# Autodesk Inventor assembly: Gas
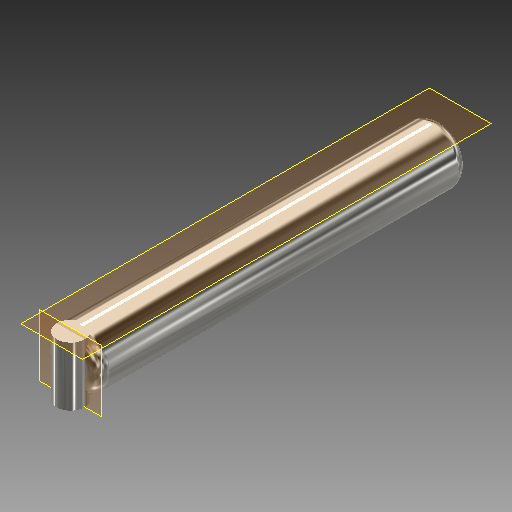
[picture p0: Inventor's stored thumbnail of the model, 512x512]
Saved by Autodesk Inventor 2021 (Build 250183000, 183)
## iProperties
Created: 2021-05-30
Part Number: Gas
Document SubType Name: Assembly
Designer: AHUJA
Author: AHUJA
## Documents named in this file (3)
- C:\Users\ahuja\Documents\Gas.iam
- F:\Files\ODM GEAR IPT\My worl\Gas Cylinder Lid.ipt
- F:\Files\ODM GEAR IPT\My worl\Gas Cylinder.ipt
## Components (2 placed, 2 different names)
1. Gas Cylinder Lid:1 — Flush:2, Mate:1
2. Gas Cylinder:1 — Flush:1, Flush:3
## Relationships (4: Flush 3, Mate 1)
- Flush:1 (12 mm): Gas Cylinder:1
- Flush:2: Gas Cylinder Lid:1
- Flush:3 (160 mm): Gas Cylinder:1
- Mate:1: Gas Cylinder Lid:1
